# Autodesk Inventor assembly: Nespresso-Assembly
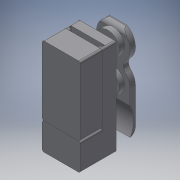
[picture p0: Inventor's stored thumbnail of the model, 180x180]
Saved by Autodesk Inventor 2017 (Build 210142000, 142)
## iProperties
Created: 2018-08-29
Part Number: Nespresso-Assembly
Document SubType Name: Assembly
Designer: 45027374
Author: 45027374
## Documents named in this file (4)
- C:\cloudstor\Documents\3Dprints\NespressoSpeedfiller\Nespresso-Assembly.iam
- C:\cloudstor\Documents\3Dprints\NespressoSpeedfiller\NespressoSpeedfiller-base.ipt
- C:\cloudstor\Documents\3Dprints\NespressoSpeedfiller\NespressoSpeedfiller.ipt
- C:\cloudstor\Documents\3Dprints\NespressoSpeedfiller\NespressoSpeedfiller-tamper.ipt
## Components (3 placed, 3 different names)
1. NespressoSpeedfiller-base:1 — Mate:1, Mate:2, Mate:3, Mate:4, Mate:5, Mate:6, Mate:7, Mate:8
2. NespressoSpeedfiller:1 — Mate:4, Mate:5, Mate:6
3. NespressoSpeedfiller-tamper:1 — Mate:7, Mate:8
## Relationships (8: Mate 8)
- Mate:1: NespressoSpeedfiller-base:1
- Mate:2: NespressoSpeedfiller-base:1
- Mate:3: NespressoSpeedfiller-base:1
- Mate:4: NespressoSpeedfiller-base:1 ↔ NespressoSpeedfiller:1
- Mate:5: NespressoSpeedfiller-base:1 ↔ NespressoSpeedfiller:1
- Mate:6: NespressoSpeedfiller-base:1 ↔ NespressoSpeedfiller:1
- Mate:7: NespressoSpeedfiller-base:1 ↔ NespressoSpeedfiller-tamper:1
- Mate:8: NespressoSpeedfiller-base:1 ↔ NespressoSpeedfiller-tamper:1
